# Autodesk Inventor assembly: hotend-new
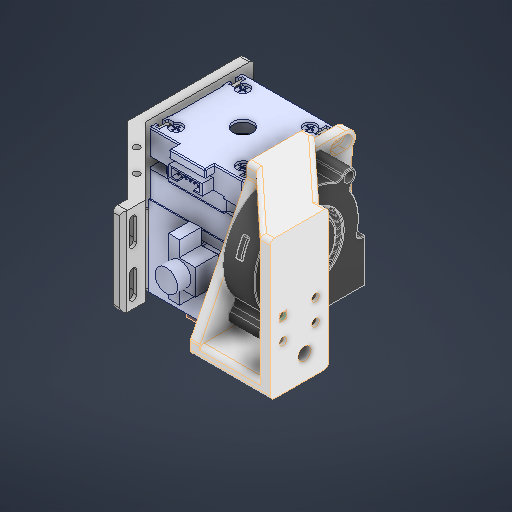
[picture p0: Inventor's stored thumbnail of the model, 512x512]
Saved by Autodesk Inventor 2025 (Build 290162000, 162)
## iProperties
Created: 2024-07-16
Part Number: hotend-new
Document SubType Name: Assembly
Designer: Windows 7 was better
Author: Windows 7 was better
## iProperties of the stored document BL-touch.ipt
Created: 2017-04-23
Part Number: BL-touch
Material: Generic
Description: STEP AP214
Document SubType Name: Modeling
Designer: Windows 7 was better
Density: 1 g/cm^3
Appearance: Default
Sending System: SolidWorks 2016
Preprocessor: SwSTEP 2.0
Title: BL-touch.STEP
Revision Number: ANY
## iProperties of the stored document Radial_Fan_50x15 v8.ipt
Created: 2022-08-24
Part Number: Radial_Fan_50x15
Material: Acier
Document SubType Name: Modeling
Designer: Windows 7 was better
Density: 7.85 g/cm^3
Appearance: Default
Sending System: Autodesk Translation Framework v11.7.0.108
Preprocessor: ST-DEVELOPER v19
Title: C:/Users/Admin/Downloads/Radial_Fan_50x15 v8.step
## Documents named in this file (12)
- C:\Users\Windows 7 was better\GitHub\ReplicatorPlusConversion\CAD\Inventor\hotend-new.iam
- C:\Users\Windows 7 was better\GitHub\ReplicatorPlusConversion\CAD\Inventor\Hemera_XS_Reference_CAD.ipt
- C:\Users\Windows 7 was better\GitHub\ReplicatorPlusConversion\CAD\Inventor\eddy.ipt
- C:\Users\Windows 7 was better\GitHub\ReplicatorPlusConversion\CAD\Inventor\the wall.ipt
- C:\Users\Windows 7 was better\GitHub\ReplicatorPlusConversion\CAD\Inventor\bolts reference.ipt
- C:\Users\Windows 7 was better\GitHub\ReplicatorPlusConversion\CAD\Inventor\hemera-xs-duct-mount-v2.ipt
- C:\Users\Windows 7 was better\GitHub\ReplicatorPlusConversion\CAD\Inventor\mount-1.ipt
- **C:\Users\Windows 7 was better\GitHub\ReplicatorPlusConversion\CAD\Inventor\hotend-new.iam*LocalDocs*xAaaaq0daAaaaaaaaAaaaq44uYf*Radial_Fan_50x15 v8.ipt
- **C:\Users\Windows 7 was better\GitHub\ReplicatorPlusConversion\CAD\Inventor\hotend-new.iam*LocalDocs*xAaaaalaaAaaaaaaaAaaaajj33h*BL-touch.ipt
- **C:\Users\Windows 7 was better\Documents\GitHub\ReplicatorPlusConversion\CAD\Inventor\hotend-new.iam*LocalDocs*xAaaaq0daAaaaaaaaAaaaq44uYf*Radial_Fan_50x15 v8.ipt
- C:\Users\Windows 7 was better\Downloads\Radial_Fan_50x15 v8.step
- C:\Users\Windows 7 was better\Downloads\BL-touch.STEP
## Components (8 placed, 8 different names)
1. Hemera_XS_Reference_CAD:1 — Flush:4
2. the wall:1
3. bolts reference:1 — Flush:3, Flush:5
4. hemera-xs-duct-mount-v2:1 — Flush:5
5. eddy:2 — Flush:6
6. mount-1:1 — Flush:3, Flush:4, Flush:6, Flush:7
7. Radial_Fan_50x15 v8:1
8. BL-touch:1 — Flush:7
## Relationships (5: Flush 5)
- Flush:3: bolts reference:1 ↔ mount-1:1
- Flush:4: Hemera_XS_Reference_CAD:1 ↔ mount-1:1
- Flush:5: bolts reference:1 ↔ hemera-xs-duct-mount-v2:1
- Flush:6: eddy:2 ↔ mount-1:1
- Flush:7: mount-1:1 ↔ BL-touch:1
